# Autodesk Inventor assembly: Intro a ensamble
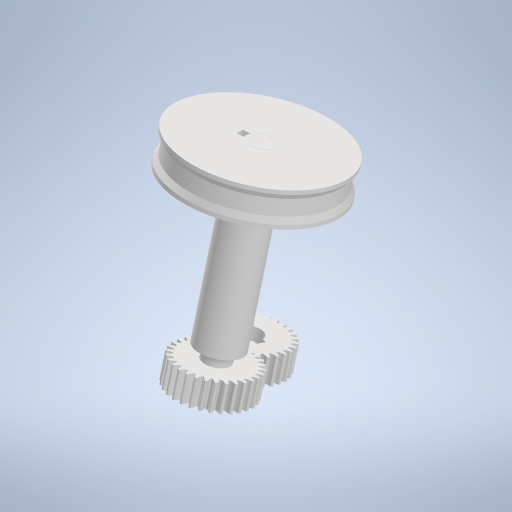
[picture p0: Inventor's stored thumbnail of the model, 512x512]
Saved by Autodesk Inventor 2024 (Build 280153000, 153)
## iProperties
Created: 2024-03-31
Part Number: Intro a ensamble
Document SubType Name: Assembly
Designer: usuario
Author: usuario
## Documents named in this file (6)
- C:\Users\usuario\Desktop\Landivar Jose\2024\Dinamica\Intro a ensamble.iam
- C:\Users\usuario\Downloads\CUÑA (3).ipt
- C:\Users\usuario\Downloads\EJE_CUÑEROS (1).ipt
- C:\Users\usuario\Downloads\POLEA (1).ipt
- C:\Users\usuario\Downloads\ENGRANE (1).ipt
- C:\Users\usuario\Downloads\ENGRANE (1)_CPY1.ipt
## Components (6 placed, 5 different names)
1. CUÑA (3):1 — Rigid:1
2. EJE_CUÑEROS (1):1 — Rigid:1, Rotational:1, Rigid:2
3. POLEA (1):1 — Rotational:1
4. ENGRANE (1):1 — Rigid:3, Rotation:1, Rotation:2, Tangent:1, Rotation:3, Flush:1, Rotation:4
5. CUÑA (3):4 — Rigid:2, Rigid:3
6. ENGRANE (1)_CPY1:1 — Rotation:1, Rotation:2, Tangent:1, Rotation:3, Flush:1, Rotation:4
## Relationships (10: RelateRotation 4, WeldJoint 3, RevoluteJoint 1, Tangent 1, Flush 1)
- Rigid:1 [WeldJoint]: CUÑA (3):1 ↔ EJE_CUÑEROS (1):1
- Rotational:1 [RevoluteJoint]: EJE_CUÑEROS (1):1 ↔ POLEA (1):1
- Rigid:2 [WeldJoint]: EJE_CUÑEROS (1):1 ↔ CUÑA (3):4
- Rigid:3 [WeldJoint]: ENGRANE (1):1 ↔ CUÑA (3):4
- Rotation:1 [RelateRotation] (1 ul): ENGRANE (1):1 ↔ ENGRANE (1)_CPY1:1
- Rotation:2 [RelateRotation] (1 ul): ENGRANE (1):1 ↔ ENGRANE (1)_CPY1:1
- Tangent:1: ENGRANE (1):1 ↔ ENGRANE (1)_CPY1:1
- Rotation:3 [RelateRotation] (1 ul): ENGRANE (1):1 ↔ ENGRANE (1)_CPY1:1
- Flush:1: ENGRANE (1):1 ↔ ENGRANE (1)_CPY1:1
- Rotation:4 [RelateRotation] (1 ul): ENGRANE (1):1 ↔ ENGRANE (1)_CPY1:1
